# Autodesk Inventor assembly: BiggerAssembly
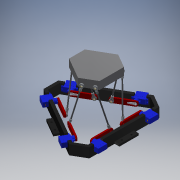
[picture p0: Inventor's stored thumbnail of the model, 180x180]
Saved by Autodesk Inventor 2018.1 (Build 221171000, 171)
## iProperties
Created: 2017-11-10
Part Number: BiggerAssembly
Document SubType Name: Assembly
Designer: sodie
Author: sodie
## Documents named in this file (8)
- C:\Users\sodie\Documents\.School Work\Year 4\MECHTRON 4TB6\Stewart Platform CAD Parts\BiggerAssembly.iam
- C:\Users\sodie\Documents\.School Work\Year 4\MECHTRON 4TB6\Stewart Platform CAD Parts\Stewart_Base.ipt
- C:\Users\sodie\Documents\.School Work\Year 4\MECHTRON 4TB6\Micro Servo CAD\Servo-MG90S.ipt
- C:\Users\sodie\Documents\.School Work\Year 4\MECHTRON 4TB6\Stewart Platform CAD Parts\Stewart_ServoArm.ipt
- C:\Users\sodie\Documents\School Work\Year 4\MECHTRON 4TB6\Micro Servo CAD\SG90 plastic Horn White.ipt
- C:\Users\sodie\Documents\.School Work\Year 4\MECHTRON 4TB6\Stewart Platform CAD Parts\Stewart_BallJoint.ipt
- C:\Users\sodie\Documents\.School Work\Year 4\MECHTRON 4TB6\Stewart Platform CAD Parts\Stewart_ThreadedRod.ipt
- C:\Users\sodie\Documents\.School Work\Year 4\MECHTRON 4TB6\Stewart_Platform_Original3.ipt
## Components (38 placed, 7 different names)
1. Stewart_Base:1 — Mate:1, Mate:2, Flush:1, Mate:3, Mate:4, Mate:5, Mate:6, Mate:7, Mate:8, Mate:9, Mate:10, Mate:11, Mate:18, Mate:19, Mate:20, Mate:21, Mate:22, Mate:23, Mate:24, Mate:25, Mate:26, Angle:13, Angle:14
2. Servo-MG90S:1 — Mate:18, Mate:19, Mate:20, Mate:39, Mate:40
3. Servo-MG90S:2 — Mate:3, Mate:4, Mate:5, Mate:41, Mate:42
4. Servo-MG90S:3 — Mate:24, Mate:25, Mate:26, Mate:43, Mate:44
5. Servo-MG90S:4 — Mate:21, Mate:22, Mate:23, Mate:45, Mate:46
6. Servo-MG90S:5 — Mate:6, Mate:7, Mate:8, Mate:49, Mate:50
7. Servo-MG90S:6 — Mate:9, Mate:10, Mate:11, Mate:47, Mate:48
8. SG90 plastic Horn White:1 — Mate:27, Mate:28, Flush:2, Mate:39, Mate:40
9. Stewart_ServoArm:1 — Mate:27, Mate:28, Flush:2, Mate:86, Flush:8
10. SG90 plastic Horn White:2 — Mate:41, Mate:42
11. Stewart_ServoArm:2 — Mate:84, Flush:8
12. SG90 plastic Horn White:3 — Mate:43
13. Stewart_ServoArm:3 — Mate:44, Mate:81, Flush:9
14. SG90 plastic Horn White:4 — Mate:45
15. Stewart_ServoArm:4 — Mate:46, Mate:85, Flush:9
16. SG90 plastic Horn White:5 — Mate:49, Mate:50
17. Stewart_ServoArm:5 — Mate:83
18. SG90 plastic Horn White:6 — Mate:47, Mate:48
19. Stewart_ServoArm:6 — Mate:89
20. Stewart_BallJoint:4 — Mate:52, Angle:2, Tangent:2, Mate:83, Angle:19
21. Stewart_BallJoint:6 — Mate:51, Angle:1, Tangent:1, Mate:92, Angle:18
22. Stewart_ThreadedRod:1 — Mate:51, Angle:1, Tangent:1, Mate:52, Angle:2, Tangent:2
23. Stewart_BallJoint:7 — Mate:89, Angle:19
24. Stewart_BallJoint:8 — Angle:17, Mate:90
25. Stewart_ThreadedRod:2
26. Stewart_BallJoint:9 — Mate:86
27. Stewart_BallJoint:10 — Mate:76
28. Stewart_ThreadedRod:3
29. Stewart_BallJoint:11 — Mate:84
30. Stewart_BallJoint:12 — Mate:93, Angle:18
31. Stewart_ThreadedRod:4
32. Stewart_BallJoint:13 — Mate:81, Angle:15
33. Stewart_BallJoint:14 — Mate:78, Angle:17
34. Stewart_ThreadedRod:5
35. Stewart_BallJoint:15 — Mate:75
36. Stewart_BallJoint:16 — Mate:85, Angle:15
37. Stewart_ThreadedRod:6
38. Stewart_Platform_Original3:1 — Mate:75, Mate:76, Mate:78, Angle:13, Angle:14, Mate:90, Mate:92, Mate:93
## Relationships (107: Mate 68, Angle 18, Tangent 12, Flush 9)
- Mate:1: Stewart_Base:1
- Mate:2: Stewart_Base:1
- Flush:1: Stewart_Base:1
- Mate:3: Stewart_Base:1 ↔ Servo-MG90S:2
- Mate:4: Stewart_Base:1 ↔ Servo-MG90S:2
- Mate:5: Stewart_Base:1 ↔ Servo-MG90S:2
- Mate:6: Stewart_Base:1 ↔ Servo-MG90S:5
- Mate:7: Stewart_Base:1 ↔ Servo-MG90S:5
- Mate:8: Stewart_Base:1 ↔ Servo-MG90S:5
- Mate:9: Stewart_Base:1 ↔ Servo-MG90S:6
- Mate:10: Stewart_Base:1 ↔ Servo-MG90S:6
- Mate:11: Stewart_Base:1 ↔ Servo-MG90S:6
- Mate:18: Stewart_Base:1 ↔ Servo-MG90S:1
- Mate:19: Stewart_Base:1 ↔ Servo-MG90S:1
- Mate:20: Stewart_Base:1 ↔ Servo-MG90S:1
- Mate:21: Stewart_Base:1 ↔ Servo-MG90S:4
- Mate:22: Stewart_Base:1 ↔ Servo-MG90S:4
- Mate:23: Stewart_Base:1 ↔ Servo-MG90S:4
- Mate:24: Stewart_Base:1 ↔ Servo-MG90S:3
- Mate:25: Stewart_Base:1 ↔ Servo-MG90S:3
- Mate:26: Stewart_Base:1 ↔ Servo-MG90S:3
- Mate:27: SG90 plastic Horn White:1 ↔ Stewart_ServoArm:1
- Mate:28: SG90 plastic Horn White:1 ↔ Stewart_ServoArm:1
- Flush:2: SG90 plastic Horn White:1 ↔ Stewart_ServoArm:1
- [Mate]: SG90 plastic Horn White:2 ↔ Stewart_ServoArm:2
- [Mate]: SG90 plastic Horn White:2 ↔ Stewart_ServoArm:2
- [Flush]: SG90 plastic Horn White:2 ↔ Stewart_ServoArm:2
- [Mate]: SG90 plastic Horn White:3 ↔ Stewart_ServoArm:3
- [Mate]: SG90 plastic Horn White:3 ↔ Stewart_ServoArm:3
- [Flush]: SG90 plastic Horn White:3 ↔ Stewart_ServoArm:3
- [Mate]: SG90 plastic Horn White:4 ↔ Stewart_ServoArm:4
- [Mate]: SG90 plastic Horn White:4 ↔ Stewart_ServoArm:4
- [Flush]: SG90 plastic Horn White:4 ↔ Stewart_ServoArm:4
- [Mate]: SG90 plastic Horn White:5 ↔ Stewart_ServoArm:5
- [Mate]: SG90 plastic Horn White:5 ↔ Stewart_ServoArm:5
- [Flush]: SG90 plastic Horn White:5 ↔ Stewart_ServoArm:5
- [Mate]: SG90 plastic Horn White:6 ↔ Stewart_ServoArm:6
- [Mate]: SG90 plastic Horn White:6 ↔ Stewart_ServoArm:6
- [Flush]: SG90 plastic Horn White:6 ↔ Stewart_ServoArm:6
- Mate:39: Servo-MG90S:1 ↔ SG90 plastic Horn White:1
- Mate:40: Servo-MG90S:1 ↔ SG90 plastic Horn White:1
- Mate:41: Servo-MG90S:2 ↔ SG90 plastic Horn White:2
- Mate:42: Servo-MG90S:2 ↔ SG90 plastic Horn White:2
- Mate:43: Servo-MG90S:3 ↔ SG90 plastic Horn White:3
- Mate:44: Servo-MG90S:3 ↔ Stewart_ServoArm:3
- Mate:45: Servo-MG90S:4 ↔ SG90 plastic Horn White:4
- Mate:46: Servo-MG90S:4 ↔ Stewart_ServoArm:4
- Mate:47: Servo-MG90S:6 ↔ SG90 plastic Horn White:6
- Mate:48: Servo-MG90S:6 ↔ SG90 plastic Horn White:6
- Mate:49: Servo-MG90S:5 ↔ SG90 plastic Horn White:5
- Mate:50: Servo-MG90S:5 ↔ SG90 plastic Horn White:5
- Mate:51: Stewart_BallJoint:6 ↔ Stewart_ThreadedRod:1
- Angle:1 (180 deg): Stewart_BallJoint:6 ↔ Stewart_ThreadedRod:1
- Tangent:1: Stewart_BallJoint:6 ↔ Stewart_ThreadedRod:1
- Mate:52: Stewart_BallJoint:4 ↔ Stewart_ThreadedRod:1
- Angle:2 (180 deg): Stewart_BallJoint:4 ↔ Stewart_ThreadedRod:1
- Tangent:2: Stewart_BallJoint:4 ↔ Stewart_ThreadedRod:1
- [Mate]: Stewart_BallJoint:8 ↔ Stewart_ThreadedRod:2
- [Angle] (180 deg): Stewart_BallJoint:8 ↔ Stewart_ThreadedRod:2
- [Tangent]: Stewart_BallJoint:8 ↔ Stewart_ThreadedRod:2
- [Mate]: Stewart_BallJoint:7 ↔ Stewart_ThreadedRod:2
- [Angle] (180 deg): Stewart_BallJoint:7 ↔ Stewart_ThreadedRod:2
- [Tangent]: Stewart_BallJoint:7 ↔ Stewart_ThreadedRod:2
- [Mate]: Stewart_BallJoint:10 ↔ Stewart_ThreadedRod:3
- [Angle] (180 deg): Stewart_BallJoint:10 ↔ Stewart_ThreadedRod:3
- [Tangent]: Stewart_BallJoint:10 ↔ Stewart_ThreadedRod:3
- [Mate]: Stewart_BallJoint:9 ↔ Stewart_ThreadedRod:3
- [Angle] (180 deg): Stewart_BallJoint:9 ↔ Stewart_ThreadedRod:3
- [Tangent]: Stewart_BallJoint:9 ↔ Stewart_ThreadedRod:3
- [Mate]: Stewart_BallJoint:12 ↔ Stewart_ThreadedRod:4
- [Angle] (180 deg): Stewart_BallJoint:12 ↔ Stewart_ThreadedRod:4
- [Tangent]: Stewart_BallJoint:12 ↔ Stewart_ThreadedRod:4
- [Mate]: Stewart_BallJoint:11 ↔ Stewart_ThreadedRod:4
- [Angle] (180 deg): Stewart_BallJoint:11 ↔ Stewart_ThreadedRod:4
- [Tangent]: Stewart_BallJoint:11 ↔ Stewart_ThreadedRod:4
- [Mate]: Stewart_BallJoint:14 ↔ Stewart_ThreadedRod:5
- [Angle] (180 deg): Stewart_BallJoint:14 ↔ Stewart_ThreadedRod:5
- [Tangent]: Stewart_BallJoint:14 ↔ Stewart_ThreadedRod:5
- [Mate]: Stewart_BallJoint:13 ↔ Stewart_ThreadedRod:5
- [Angle] (180 deg): Stewart_BallJoint:13 ↔ Stewart_ThreadedRod:5
- [Tangent]: Stewart_BallJoint:13 ↔ Stewart_ThreadedRod:5
- [Mate]: Stewart_BallJoint:16 ↔ Stewart_ThreadedRod:6
- [Angle] (180 deg): Stewart_BallJoint:16 ↔ Stewart_ThreadedRod:6
- [Tangent]: Stewart_BallJoint:16 ↔ Stewart_ThreadedRod:6
- [Mate]: Stewart_BallJoint:15 ↔ Stewart_ThreadedRod:6
- [Angle] (180 deg): Stewart_BallJoint:15 ↔ Stewart_ThreadedRod:6
- [Tangent]: Stewart_BallJoint:15 ↔ Stewart_ThreadedRod:6
- Mate:75: Stewart_BallJoint:15 ↔ Stewart_Platform_Original3:1
- Mate:76: Stewart_BallJoint:10 ↔ Stewart_Platform_Original3:1
- Mate:78: Stewart_BallJoint:14 ↔ Stewart_Platform_Original3:1
- Mate:81: Stewart_ServoArm:3 ↔ Stewart_BallJoint:13
- Mate:83: Stewart_ServoArm:5 ↔ Stewart_BallJoint:4
- Mate:84: Stewart_ServoArm:2 ↔ Stewart_BallJoint:11
- Mate:85: Stewart_ServoArm:4 ↔ Stewart_BallJoint:16
- Mate:86: Stewart_ServoArm:1 ↔ Stewart_BallJoint:9
- Angle:13 (0 deg): Stewart_Base:1 ↔ Stewart_Platform_Original3:1
- Angle:14 (0 deg): Stewart_Base:1 ↔ Stewart_Platform_Original3:1
- Flush:8: Stewart_ServoArm:1 ↔ Stewart_ServoArm:2
- Flush:9: Stewart_ServoArm:3 ↔ Stewart_ServoArm:4
- Mate:89: Stewart_ServoArm:6 ↔ Stewart_BallJoint:7
- Angle:15 (180 deg): Stewart_BallJoint:13 ↔ Stewart_BallJoint:16
- Angle:17 (0 deg): Stewart_BallJoint:8 ↔ Stewart_BallJoint:14
- Mate:90: Stewart_BallJoint:8 ↔ Stewart_Platform_Original3:1
- Mate:92: Stewart_BallJoint:6 ↔ Stewart_Platform_Original3:1
- Mate:93: Stewart_BallJoint:12 ↔ Stewart_Platform_Original3:1
- Angle:18 (0 deg): Stewart_BallJoint:6 ↔ Stewart_BallJoint:12
- Angle:19 (0 deg): Stewart_BallJoint:4 ↔ Stewart_BallJoint:7
## Named parameters: d116_d113 = 0 mm, d117_d114 = 0 mm, d118_d115 = 0 mm, d119_d113 = 0 mm, d120_d114 = 0 mm, d121_d115 = 0 mm, d122_d116_d113 = 0 mm, d123_d117_d114 = 0 mm, d124_d118_d115 = 0 mm, d125_d113 = 0 mm, d126_d114 = 0 mm, d127_d115 = 0 mm, d128_d116_d113 = 0 mm, d129_d117_d114 = 0 mm, d130_d118_d115 = 0 mm, d149_d143 = 0 mm, d150_d144 = 180 deg, d151_d145 = 0 mm, d152_d146 = 0 mm, d153_d147 = 180 deg, d154_d148 = 0 mm, d155_d143 = 0 mm, d156_d144 = 180 deg, d157_d145 = 0 mm, d158_d146 = 0 mm, d159_d147 = 180 deg, d160_d148 = 0 mm, d161_d143 = 0 mm, d162_d144 = 180 deg, d163_d145 = 0 mm, d164_d146 = 0 mm, d165_d147 = 180 deg, d166_d148 = 0 mm, d167_d143 = 0 mm, d168_d144 = 180 deg, d169_d145 = 0 mm, d170_d146 = 0 mm, d171_d147 = 180 deg, d172_d148 = 0 mm, d173_d143 = 0 mm, d174_d144 = 180 deg, d175_d145 = 0 mm, d176_d146 = 0 mm, d177_d147 = 180 deg, d178_d148 = 0 mm
